# Autodesk Inventor assembly: Double sided license plate
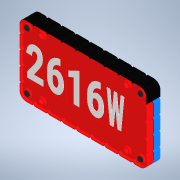
[picture p0: Inventor's stored thumbnail of the model, 180x180]
Saved by Autodesk Inventor 2022.2 (Build 262287010, 287A)
## iProperties
Created: 2022-06-18
Part Number: Double sided license plate
Document SubType Name: Assembly
Designer: Main Account
Author: Main Account
## Documents named in this file (6)
- D:\Documents\Inventor\VEX\Custom Library\Double sided license plate.iam
- D:\Documents\Inventor\VEX\Library Backup\Library 1.3\Structure\Hardware\VEX IQ Pin.ipt
- D:\Documents\Inventor\VEX\Custom Library\License Plate Numbers.ipt
- License Plate Numbers.ipt
- D:\Documents\Inventor\VEX\Custom Library\Blue License Plate Black Top.ipt
- D:\Documents\Inventor\VEX\Custom Library\Red License Plate Black Top.ipt
## Components (8 placed, 4 different names)
1. Red License Plate Black Top:1 — Insert:1, Insert:2, Insert:3, Insert:4, Mate:6, Mate:7, Mate:8
2. Blue License Plate Black Top:1 — Insert:5, Insert:6, Insert:7, Insert:8, Mate:9, Mate:10, Mate:11
3. VEX IQ Pin:1 — Insert:2, Insert:5
4. VEX IQ Pin:2 — Insert:3, Insert:8
5. VEX IQ Pin:3 — Insert:1, Insert:7
6. VEX IQ Pin:4 — Insert:4, Insert:6
7. License Plate Numbers:1 — Mate:6, Mate:7, Mate:8
8. License Plate Numbers:2 — Mate:9, Mate:10, Mate:11
## Relationships (14: Insert 8, Mate 6)
- Insert:1: Red License Plate Black Top:1 ↔ VEX IQ Pin:3
- Insert:2: Red License Plate Black Top:1 ↔ VEX IQ Pin:1
- Insert:3: Red License Plate Black Top:1 ↔ VEX IQ Pin:2
- Insert:4: Red License Plate Black Top:1 ↔ VEX IQ Pin:4
- Insert:5: Blue License Plate Black Top:1 ↔ VEX IQ Pin:1
- Insert:6: Blue License Plate Black Top:1 ↔ VEX IQ Pin:4
- Insert:7: Blue License Plate Black Top:1 ↔ VEX IQ Pin:3
- Insert:8: Blue License Plate Black Top:1 ↔ VEX IQ Pin:2
- Mate:6: Red License Plate Black Top:1 ↔ License Plate Numbers:1
- Mate:7: Red License Plate Black Top:1 ↔ License Plate Numbers:1
- Mate:8: Red License Plate Black Top:1 ↔ License Plate Numbers:1
- Mate:9: Blue License Plate Black Top:1 ↔ License Plate Numbers:2
- Mate:10: Blue License Plate Black Top:1 ↔ License Plate Numbers:2
- Mate:11: Blue License Plate Black Top:1 ↔ License Plate Numbers:2
